# Autodesk Inventor assembly: Передача клиновым ремнем1_MIR
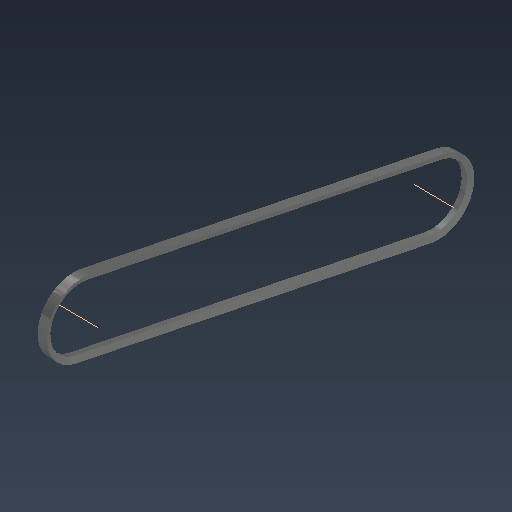
[picture p0: Inventor's stored thumbnail of the model, 512x512]
Saved by Autodesk Inventor 2026 (Build 300175000, 175)
## iProperties
Created: 2026-01-10
Part Number: Передача клиновым ремнем1_MIR
Document SubType Name: Assembly
Designer: GameHD
Author: GameHD
## Documents named in this file (2)
- C:\Users\GameHD\Desktop\Phantom 16950\шутер\Мастер проектирования\Передача клиновым ремнем1_MIR.iam
- C:\Users\GameHD\Desktop\Phantom 16950\шутер\Мастер проектирования\Клиновой ремень1_MIR.ipt
## Components (1 placed, 1 different names)
1. Клиновой ремень1_MIR:1
## Component patterns: (1 elements, first: Клиновой ремень1_MIR:1)
